# Autodesk Inventor assembly: Basic Horiozontal Assembly
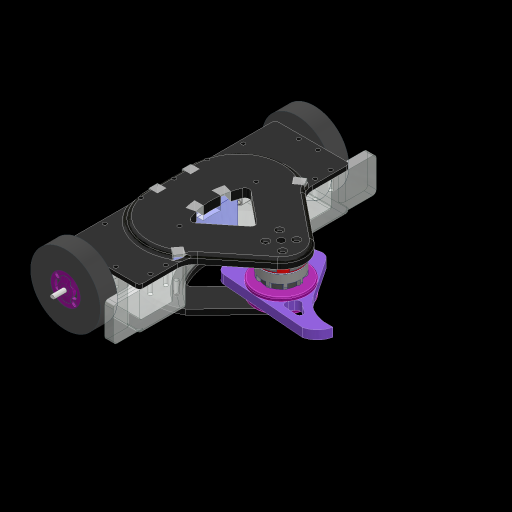
[picture p0: Inventor's stored thumbnail of the model, 512x512]
Saved by Autodesk Inventor 2023 (Build 270158000, 158)
## iProperties
Created: 2022-07-28
Part Number: Basic Horiozontal Assembly
Document SubType Name: Assembly
Designer: tandu
Mass: 412.535 g
Surface Area: 1212.79 cm^2
Volume: 278.045 cm^3
Density: 1.4837 g/cm^3
Author: tandu
## Documents named in this file (12)
- C:\Users\tandu\Documents\GrabCAD\Backup Antweights\Basic Horizontal\Basic Horiozontal Assembly.iam
- C:\Users\tandu\Documents\GrabCAD\Backup Antweights\Basic Horizontal\Horizontal TPU 22 Chassis.ipt
- C:\Users\tandu\Documents\GrabCAD\Backup Antweights\Basic Horizontal\BatteryMockup.ipt
- C:\Users\tandu\Documents\GrabCAD\Backup Antweights\Basic Horizontal\CorrectSizeWheelsIThink.ipt
- C:\Users\tandu\Documents\GrabCAD\Backup Antweights\Basic Horizontal\EMax RS2205 v1.ipt
- C:\Users\tandu\Documents\GrabCAD\Backup Antweights\Basic Horizontal\FingerTech_Silver_Spark_223350.ipt
- C:\Users\tandu\Documents\GrabCAD\Backup Antweights\Basic Horizontal\Insomnia1ToothWeapon_10_5_21.ipt
- C:\Users\tandu\Documents\GrabCAD\Backup Antweights\Basic Horizontal\BearingUpright.ipt
- C:\Users\tandu\Documents\GrabCAD\Backup Antweights\Basic Horizontal\LidAndMotorUpright.ipt
- C:\Users\tandu\Documents\GrabCAD\Backup Antweights\Basic Horizontal\57155K571_Flanged Ball Bearing.ipt
- C:\Users\tandu\Documents\GrabCAD\Backup Antweights\Basic Horizontal\New Hub for old blade.ipt
- C:\Users\tandu\Documents\GrabCAD\Backup Antweights\Basic Horizontal\New Hub for old blade Lid.ipt
## Components (13 placed, 11 different names)
1. Horizontal TPU 22 Chassis:1 — Insert:2, Mate:6, Insert:3, Mate:7, Insert:4, Insert:5, Mate:11, Mate:14, Angle:1, Angle:2, Mate:16, Flush:1, Flush:2, Flush:3, Mate:18, Mate:19
2. BatteryMockup:1 — Mate:18, Mate:19
3. CorrectSizeWheelsIThink:1 — Insert:4
4. EMax RS2205 v1:1 — Mate:4, Insert:6, Mate:17, Insert:9
5. FingerTech_Silver_Spark_223350:1 — Insert:2, Mate:6
6. Insomnia1ToothWeapon_10_5_21:1 — Mate:11, Insert:6, Insert:8, Insert:10
7. BearingUpright:1 — Mate:4, Mate:14, Angle:1, Insert:7, Flush:3
8. LidAndMotorUpright:1 — Angle:2, Mate:16, Mate:17, Insert:9, Flush:1, Flush:2
9. FingerTech_Silver_Spark_223350:2 — Insert:3, Mate:7
10. CorrectSizeWheelsIThink:2 — Insert:5
11. 57155K571_Flanged Ball Bearing:1 — Insert:7
12. New Hub for old blade:1 — Insert:8
13. New Hub for old blade Lid:1 — Insert:10
## Relationships (23: Mate 9, Insert 9, Flush 3, Angle 2)
- Mate:4: EMax RS2205 v1:1 ↔ BearingUpright:1
- Insert:2: Horizontal TPU 22 Chassis:1 ↔ FingerTech_Silver_Spark_223350:1
- Mate:6: Horizontal TPU 22 Chassis:1 ↔ FingerTech_Silver_Spark_223350:1
- Insert:3: Horizontal TPU 22 Chassis:1 ↔ FingerTech_Silver_Spark_223350:2
- Mate:7: Horizontal TPU 22 Chassis:1 ↔ FingerTech_Silver_Spark_223350:2
- Insert:4: Horizontal TPU 22 Chassis:1 ↔ CorrectSizeWheelsIThink:1
- Insert:5: Horizontal TPU 22 Chassis:1 ↔ CorrectSizeWheelsIThink:2
- Mate:11: Horizontal TPU 22 Chassis:1 ↔ Insomnia1ToothWeapon_10_5_21:1
- Insert:6 (2.54 mm): EMax RS2205 v1:1 ↔ Insomnia1ToothWeapon_10_5_21:1
- Mate:14: Horizontal TPU 22 Chassis:1 ↔ BearingUpright:1
- Angle:1 (0 deg): Horizontal TPU 22 Chassis:1 ↔ BearingUpright:1
- Angle:2 (0 deg): Horizontal TPU 22 Chassis:1 ↔ LidAndMotorUpright:1
- Insert:7: BearingUpright:1 ↔ 57155K571_Flanged Ball Bearing:1
- Insert:8: Insomnia1ToothWeapon_10_5_21:1 ↔ New Hub for old blade:1
- Mate:16: Horizontal TPU 22 Chassis:1 ↔ LidAndMotorUpright:1
- Mate:17: EMax RS2205 v1:1 ↔ LidAndMotorUpright:1
- Insert:9: EMax RS2205 v1:1 ↔ LidAndMotorUpright:1
- Insert:10: Insomnia1ToothWeapon_10_5_21:1 ↔ New Hub for old blade Lid:1
- Flush:1: Horizontal TPU 22 Chassis:1 ↔ LidAndMotorUpright:1
- Flush:2: Horizontal TPU 22 Chassis:1 ↔ LidAndMotorUpright:1
- Flush:3: Horizontal TPU 22 Chassis:1 ↔ BearingUpright:1
- Mate:18: Horizontal TPU 22 Chassis:1 ↔ BatteryMockup:1
- Mate:19: Horizontal TPU 22 Chassis:1 ↔ BatteryMockup:1
